# Autodesk Inventor assembly: SAFRS-A-0011
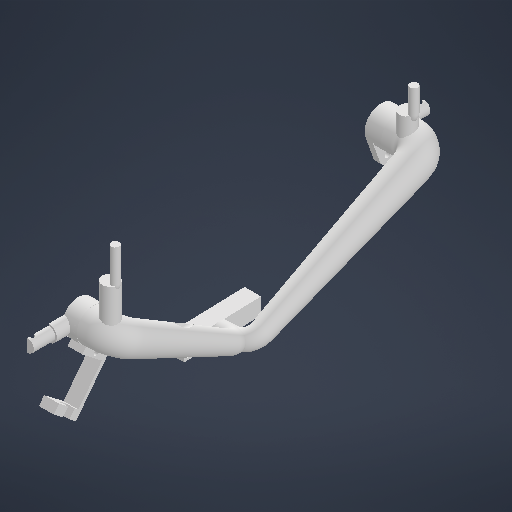
[picture p0: Inventor's stored thumbnail of the model, 512x512]
Saved by Autodesk Inventor 2026.2 (Build 302298000, 298)
## iProperties
Created: 2025-11-28
Part Number: SAFRS-A-0011
Document SubType Name: Assembly
Designer: jaewook
Author: jaewook
Title: Roll Support Right Assembly
## Documents named in this file (3)
- C:\Users\jk000\OneDrive\Desktop\git\SAFRS\mechanical\inventor\02__subassemblies\roll_support_right.iam
- C:\Users\jk000\OneDrive\Desktop\git\SAFRS\mechanical\inventor\01_parts\roll_rear_v1.ipt
- C:\Users\jk000\OneDrive\Desktop\git\SAFRS\mechanical\inventor\01_parts\base_rear.ipt
## Components (2 placed, 2 different names)
1. roll_rear_v1:2 — 메이트:1
2. base_rear:1 — 메이트:1
## Relationships (1: Mate 1)
- 메이트:1 [Mate]: roll_rear_v1:2 ↔ base_rear:1
